# Autodesk Inventor assembly: Intake Assembly
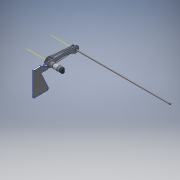
[picture p0: Inventor's stored thumbnail of the model, 180x180]
Saved by Autodesk Inventor 2019.4 (Build 234330000, 330)
## iProperties
Created: 2020-01-05
Part Number: Intake Assembly
Document SubType Name: Assembly
Designer: admin
Author: admin
## Documents named in this file (7)
- C:\Users\admin\Desktop\FRC 2020 Engineering\GitHub\7738-2020\Intake Mechanism\Intake Assembly.iam
- C:\Users\admin\Desktop\FRC 2020 Engineering\GitHub\7738-2020\Intake Mechanism\Main Axle.ipt
- C:\Users\admin\Desktop\FRC 2020 Engineering\GitHub\7738-2020\Intake Mechanism\Intake Arm Left.ipt
- C:\Users\admin\Desktop\FRC 2020 Engineering\GitHub\7738-2020\CAD\Gearbox\F6800.ipt
- C:\Users\admin\Desktop\FRC 2020 Engineering\GitHub\7738-2020\Intake Mechanism\Neverest\am-3103 NeveRest 60.ipt
- C:\Users\admin\Desktop\FRC 2020 Engineering\GitHub\7738-2020\Intake Mechanism\Intake Assembly\Design Accelerator\Synchronous Belts Transmission1.iam
- C:\Users\admin\Desktop\FRC 2020 Engineering\GitHub\7738-2020\Intake Mechanism\Intake Mount.ipt
## Components (7 placed, 6 different names)
1. Main Axle:1 — Mate:9, Flush:2
2. Intake Arm Left:1 — Mate:1, Mate:2, Mate:3, Mate:4, Mate:6, Mate:7, Flush:1, Mate:8, Angle:1
3. F6800:1 — Mate:1, Mate:4, Mate:9
4. F6800:2 — Mate:2, Mate:3, Mate:10, Mate:11
5. am-3103 NeveRest 60:1 — Mate:6, Mate:7, Mate:8
6. Synchronous Belts Transmission:1 [sub-assembly] — Flush:2
7. Intake Mount:1 — Mate:10, Mate:11, Angle:1
## Relationships (13: Mate 10, Flush 2, Angle 1)
- Mate:1: Intake Arm Left:1 ↔ F6800:1
- Mate:2: Intake Arm Left:1 ↔ F6800:2
- Mate:3 (0.2 mm): Intake Arm Left:1 ↔ F6800:2
- Mate:4 (0.2 mm): Intake Arm Left:1 ↔ F6800:1
- Mate:6: Intake Arm Left:1 ↔ am-3103 NeveRest 60:1
- Mate:7 (0.2 mm): Intake Arm Left:1 ↔ am-3103 NeveRest 60:1
- Flush:1 (-25 mm): Intake Arm Left:1
- Mate:8: Intake Arm Left:1 ↔ am-3103 NeveRest 60:1
- Mate:9: Main Axle:1 ↔ F6800:1
- Flush:2: Main Axle:1 ↔ Synchronous Belts Transmission:1
- Mate:10: F6800:2 ↔ Intake Mount:1
- Mate:11 (1.1 mm): F6800:2 ↔ Intake Mount:1
- Angle:1 (0 deg): Intake Arm Left:1 ↔ Intake Mount:1
